# Autodesk Inventor assembly: Camera-Holder
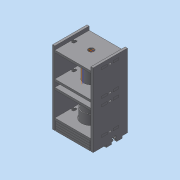
[picture p0: Inventor's stored thumbnail of the model, 180x180]
Saved by Autodesk Inventor 2016 SP1 (Build 200210100, 210)
## iProperties
Created: 2016-01-24
Part Number: Camera-Holder
Document SubType Name: Assembly
Designer: Mohamed A.
Author: Mohamed A.
## Documents named in this file (17)
- C:\Users\Mohamed\Documents\inventor\StemCellsPlatform\Laser Cut\Camera-Holder\Camera-Holder.iam
- C:\Users\Mohamed\Documents\inventor\StemCellsPlatform\Laser Cut\Camera-Holder\Camera-Holder_Front.ipt
- C:\Users\Mohamed\Documents\inventor\StemCellsPlatform\Bearings\LM8UU 8mm Linear Bearing.ipt
- C:\Users\Mohamed\Documents\inventor\StemCellsPlatform\Laser Cut\Camera-Holder\Camera-Holder_Top.ipt
- C:\Users\Mohamed\Documents\inventor\StemCellsPlatform\Camera\Raspberry Pi Camera rev 1.3\RasPi_Camera.iam
- C:\Users\Mohamed\Documents\inventor\StemCellsPlatform\Laser Cut\Camera-Holder\Camera-Holder_Camera-Base.ipt
- C:\Users\Mohamed\Documents\inventor\StemCellsPlatform\Lead Screws\8mm flanged lead screw nut with 2mm thread.ipt
- C:\Users\Mohamed\Documents\inventor\StemCellsPlatform\Laser Cut\Camera-Holder\Camera-Holder_Side.ipt
- C:\Users\Mohamed\Documents\inventor\StemCellsPlatform\Fasters\ISO 7045 - M3 x 16 - 4.8 - H - ISO1- Straight.ipt
- ISO 7045 - M3 x 16 - 4.8 - H - ISO1.ipt
- C:\Users\Mohamed\Documents\inventor\StemCellsPlatform\Laser Cut\Camera-Holder\Camera-Holder_Bearing-Ring-Outer-Right.ipt
- C:\Users\Mohamed\Documents\inventor\StemCellsPlatform\Laser Cut\Camera-Holder\Camera-Holder_Bearing-Ring-Middle-Right.ipt
- C:\Users\Mohamed\Documents\inventor\StemCellsPlatform\Laser Cut\Camera-Holder\Camera-Holder_Bearing-Ring-Outer-Left.ipt
- C:\Users\Mohamed\Documents\inventor\StemCellsPlatform\Laser Cut\Camera-Holder\Camera-Holder_Bearing-Ring-Middle-Left.ipt
- C:\Users\Mohamed\Documents\inventor\StemCellsPlatform\Laser Cut\Camera-Holder\Camera-Holder_Bearing-Side.ipt
- C:\Users\Mohamed\Documents\inventor\StemCellsPlatform\Boards\Raspberry Pi Camera rev 1.3\RaspberryPi2 STEP214.iam
- C:\Users\Mohamed\Documents\inventor\StemCellsPlatform\Camera\new\Assembly1.iam
## Components (25 placed, 15 different names)
1. Camera-Holder_Front:1 — Flush:1, Flush:5, Flush:14, Flush:23, Flush:24, Flush:29, Mate:9, Mate:10
2. Camera-Holder_Front:2 — Flush:3, Flush:11, Insert:5, Insert:6, Flush:17, Flush:20, Flush:18, Flush:28, Flush:40, Mate:16, Mate:17, Mate:18, Mate:20
3. LM8UU 8mm Linear Bearing:1 — Mate:21, Mate:22
4. LM8UU 8mm Linear Bearing:2 — Tangent:4, Mate:4, Mate:5
5. Camera-Holder_Bearing-Ring-Middle-Right:1 — Flush:30, Flush:31, Mate:11
6. Camera-Holder_Bearing-Ring-Middle-Left:1 — Flush:38, Flush:39, Mate:15
7. Camera-Holder_Top:1 — Mate:1, Mate:2, Mate:3, Flush:19, Flush:21, Flush:22, Flush:26, Flush:27, Flush:29, Mate:9, Mate:10, Flush:31, Flush:32, Flush:34, Flush:36, Flush:38, Flush:40, Mate:16, Mate:17, Flush:41, Mate:19, Mate:23
8. RasPi_Camera:1 [sub-assembly] — Mate:1, Mate:2, Mate:3, Insert:2, Insert:3, Insert:4
9. Camera-Holder_Camera-Base:1
10. Camera-Holder_Bearing-Ring-Outer-Left:2 — Mate:4, Mate:5, Flush:12, Flush:41, Mate:19
11. Camera-Holder_Bearing-Ring-Outer-Left:1 — Flush:36, Flush:37, Mate:14
12. Camera-Holder_Bearing-Ring-Outer-Right:2 — Flush:34, Flush:35, Mate:13
13. Camera-Holder_Bearing-Ring-Outer-Right:1 — Flush:16, Flush:25, Flush:32, Flush:33, Mate:12, Mate:21, Mate:22
14. 8mm flanged lead screw nut with 2mm thread:1 — Insert:5, Insert:6
15. Camera-Holder_Side:1 — Flush:11, Flush:18, Flush:19, Flush:20, Flush:37, Mate:14, Flush:39, Mate:15
16. Camera-Holder_Bearing-Side:2 — Tangent:2, Flush:5, Tangent:4, Flush:12, Flush:27, Flush:28, Mate:18
17. Camera-Holder_Bearing-Side:1 — Flush:1, Tangent:1, Flush:3, Flush:26, Mate:20
18. Camera-Holder_Side:4 — Flush:22, Flush:23, Flush:24, Flush:30, Mate:11, Flush:33, Mate:12, Flush:35, Mate:13
19. ISO 7045 - M3 x 16 - 4.8 - H - ISO1:7 — Insert:2, Mate:24
20. ISO 7045 - M3 x 16 - 4.8 - H - ISO1:8 — Insert:3, Tangent:2, Mate:25
21. ISO 7045 - M3 x 16 - 4.8 - H - ISO1:5 — Insert:4, Tangent:1
22. ISO 7045 - M3 x 16 - 4.8 - H - ISO1:6 — Mate:26, Mate:27
23. Camera-Holder_Top:2 — Flush:14, Flush:16, Flush:17, Flush:21, Flush:25, Mate:6, Mate:7, Mate:8
24. RaspberryPi2 STEP214:1 [sub-assembly] — Mate:6, Mate:7, Mate:8
25. Assembly1:1 [sub-assembly] — Mate:23, Mate:24, Mate:25, Mate:26, Mate:27
## Relationships (67: Flush 32, Mate 27, Insert 5, Tangent 3)
- Mate:1: Camera-Holder_Top:1 ↔ RasPi_Camera:1
- Mate:2: Camera-Holder_Top:1 ↔ RasPi_Camera:1
- Mate:3: Camera-Holder_Top:1 ↔ RasPi_Camera:1
- Insert:2 (3 mm): RasPi_Camera:1 ↔ ISO 7045 - M3 x 16 - 4.8 - H - ISO1:7
- Insert:3 (3 mm): RasPi_Camera:1 ↔ ISO 7045 - M3 x 16 - 4.8 - H - ISO1:8
- Insert:4 (3 mm): RasPi_Camera:1 ↔ ISO 7045 - M3 x 16 - 4.8 - H - ISO1:5
- Flush:1: Camera-Holder_Front:1 ↔ Camera-Holder_Bearing-Side:1
- Tangent:1 (1 mm): Camera-Holder_Bearing-Side:1 ↔ ISO 7045 - M3 x 16 - 4.8 - H - ISO1:5
- Flush:3: Camera-Holder_Front:2 ↔ Camera-Holder_Bearing-Side:1
- Tangent:2 (1 mm): Camera-Holder_Bearing-Side:2 ↔ ISO 7045 - M3 x 16 - 4.8 - H - ISO1:8
- Flush:5: Camera-Holder_Front:1 ↔ Camera-Holder_Bearing-Side:2
- Tangent:4 (7 mm): LM8UU 8mm Linear Bearing:2 ↔ Camera-Holder_Bearing-Side:2
- Flush:11: Camera-Holder_Front:2 ↔ Camera-Holder_Side:1
- Mate:4: LM8UU 8mm Linear Bearing:2 ↔ Camera-Holder_Bearing-Ring-Outer-Left:2
- Mate:5: LM8UU 8mm Linear Bearing:2 ↔ Camera-Holder_Bearing-Ring-Outer-Left:2
- Flush:12: Camera-Holder_Bearing-Ring-Outer-Left:2 ↔ Camera-Holder_Bearing-Side:2
- Flush:14: Camera-Holder_Front:1 ↔ Camera-Holder_Top:2
- Insert:5: Camera-Holder_Front:2 ↔ 8mm flanged lead screw nut with 2mm thread:1
- Insert:6: Camera-Holder_Front:2 ↔ 8mm flanged lead screw nut with 2mm thread:1
- Flush:16: Camera-Holder_Bearing-Ring-Outer-Right:1 ↔ Camera-Holder_Top:2
- Flush:17: Camera-Holder_Front:2 ↔ Camera-Holder_Top:2
- Flush:18 (5 mm): Camera-Holder_Front:2 ↔ Camera-Holder_Side:1
- Flush:19: Camera-Holder_Top:1 ↔ Camera-Holder_Side:1
- Flush:20: Camera-Holder_Front:2 ↔ Camera-Holder_Side:1
- Flush:21: Camera-Holder_Top:1 ↔ Camera-Holder_Top:2
- Flush:22: Camera-Holder_Top:1 ↔ Camera-Holder_Side:4
- Flush:23: Camera-Holder_Front:1 ↔ Camera-Holder_Side:4
- Flush:24 (5 mm): Camera-Holder_Front:1 ↔ Camera-Holder_Side:4
- Flush:25: Camera-Holder_Bearing-Ring-Outer-Right:1 ↔ Camera-Holder_Top:2
- Flush:26: Camera-Holder_Top:1 ↔ Camera-Holder_Bearing-Side:1
- Flush:27: Camera-Holder_Top:1 ↔ Camera-Holder_Bearing-Side:2
- Flush:28: Camera-Holder_Front:2 ↔ Camera-Holder_Bearing-Side:2
- Mate:6 (15 mm): Camera-Holder_Top:2 ↔ RaspberryPi2 STEP214:1
- Mate:7: Camera-Holder_Top:2 ↔ RaspberryPi2 STEP214:1
- Mate:8: Camera-Holder_Top:2 ↔ RaspberryPi2 STEP214:1
- Flush:29: Camera-Holder_Front:1 ↔ Camera-Holder_Top:1
- Mate:9: Camera-Holder_Front:1 ↔ Camera-Holder_Top:1
- Mate:10: Camera-Holder_Front:1 ↔ Camera-Holder_Top:1
- Flush:30: Camera-Holder_Bearing-Ring-Middle-Right:1 ↔ Camera-Holder_Side:4
- Flush:31: Camera-Holder_Bearing-Ring-Middle-Right:1 ↔ Camera-Holder_Top:1
- Mate:11: Camera-Holder_Bearing-Ring-Middle-Right:1 ↔ Camera-Holder_Side:4
- Flush:32: Camera-Holder_Top:1 ↔ Camera-Holder_Bearing-Ring-Outer-Right:1
- Flush:33: Camera-Holder_Bearing-Ring-Outer-Right:1 ↔ Camera-Holder_Side:4
- Mate:12: Camera-Holder_Bearing-Ring-Outer-Right:1 ↔ Camera-Holder_Side:4
- Flush:34: Camera-Holder_Top:1 ↔ Camera-Holder_Bearing-Ring-Outer-Right:2
- Flush:35: Camera-Holder_Bearing-Ring-Outer-Right:2 ↔ Camera-Holder_Side:4
- Mate:13: Camera-Holder_Bearing-Ring-Outer-Right:2 ↔ Camera-Holder_Side:4
- Flush:36: Camera-Holder_Top:1 ↔ Camera-Holder_Bearing-Ring-Outer-Left:1
- Flush:37: Camera-Holder_Bearing-Ring-Outer-Left:1 ↔ Camera-Holder_Side:1
- Mate:14: Camera-Holder_Bearing-Ring-Outer-Left:1 ↔ Camera-Holder_Side:1
- Flush:38: Camera-Holder_Bearing-Ring-Middle-Left:1 ↔ Camera-Holder_Top:1
- Flush:39: Camera-Holder_Bearing-Ring-Middle-Left:1 ↔ Camera-Holder_Side:1
- Mate:15: Camera-Holder_Bearing-Ring-Middle-Left:1 ↔ Camera-Holder_Side:1
- Flush:40: Camera-Holder_Front:2 ↔ Camera-Holder_Top:1
- Mate:16: Camera-Holder_Front:2 ↔ Camera-Holder_Top:1
- Mate:17: Camera-Holder_Front:2 ↔ Camera-Holder_Top:1
- Mate:18: Camera-Holder_Front:2 ↔ Camera-Holder_Bearing-Side:2
- Flush:41: Camera-Holder_Top:1 ↔ Camera-Holder_Bearing-Ring-Outer-Left:2
- Mate:19: Camera-Holder_Top:1 ↔ Camera-Holder_Bearing-Ring-Outer-Left:2
- Mate:20: Camera-Holder_Front:2 ↔ Camera-Holder_Bearing-Side:1
- Mate:21: LM8UU 8mm Linear Bearing:1 ↔ Camera-Holder_Bearing-Ring-Outer-Right:1
- Mate:22: LM8UU 8mm Linear Bearing:1 ↔ Camera-Holder_Bearing-Ring-Outer-Right:1
- Mate:23: Camera-Holder_Top:1 ↔ Assembly1:1
- Mate:24: ISO 7045 - M3 x 16 - 4.8 - H - ISO1:7 ↔ Assembly1:1
- Mate:25: ISO 7045 - M3 x 16 - 4.8 - H - ISO1:8 ↔ Assembly1:1
- Mate:26: ISO 7045 - M3 x 16 - 4.8 - H - ISO1:6 ↔ Assembly1:1
- Mate:27: ISO 7045 - M3 x 16 - 4.8 - H - ISO1:6 ↔ Assembly1:1
